# Autodesk Inventor assembly: OBG-Gehäuse
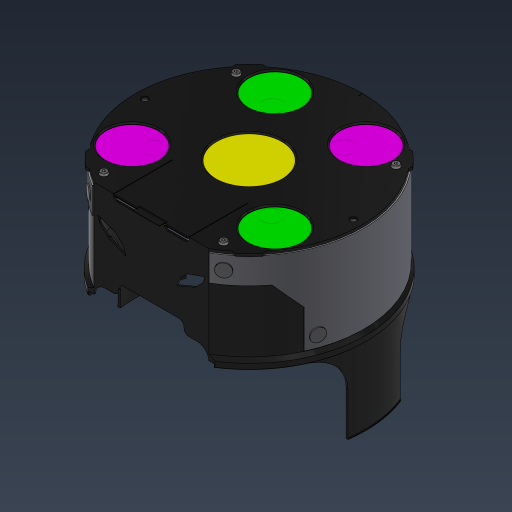
[picture p0: Inventor's stored thumbnail of the model, 512x512]
Saved by Autodesk Inventor 2023.1 (Build 271208000, 208)
## iProperties
Part Number: OBG-Gehäuse
Material: Generisch
Document SubType Name: Assembly
Designer: rYan
Mass: 129.127 g
Surface Area: 1997.42 cm^2
Volume: 130.879 cm^3
Density: 0.986618 g/cm^3
Author: rYan
## Documents named in this file (8)
- D:\TIGERsGIT\Hardware\mechanik\2024\Inventor\Robot\Case\OBG-Gehäuse.iam
- D:\TIGERsGIT\Hardware\mechanik\2024\Inventor\Robot\Case\Gehäuse Unterplatte.ipt
- D:\TIGERsGIT\Hardware\mechanik\2024\Inventor\Purchased Parts\Papier 40mm.ipt
- D:\TIGERsGIT\Hardware\mechanik\2024\Inventor\Inhaltscenter\de-DE\DIN 7984\DIN 7984 - M3 x 5.ipt
- D:\TIGERsGIT\Hardware\mechanik\2024\Inventor\Purchased Parts\Papier Teamfarbe.ipt
- D:\TIGERsGIT\Hardware\mechanik\2024\Inventor\Robot\Case\Gehäuse Mantel.ipt
- D:\TIGERsGIT\Hardware\mechanik\2024\Inventor\Robot\Case\Gehäuse Schnappfolie.ipt
- D:\TIGERsGIT\Hardware\mechanik\2024\Inventor\Robot\Case\Druckknopf.ipt
## Components (17 placed, 7 different names)
1. Gehäuse Mantel magnetisch:1 — Passend:9, Passend:10, Fluchtend:6, Einfügen:1, Einfügen:2, Einfügen:3, Einfügen:4, Passend:17, Einfügen:5, Einfügen:6, Einfügen:7, Einfügen:8, Einfügen:9, Passend:20
2. Gehäuse Unterplatte:1 — Einfügen:9, Fluchtend:7
3. Gehäuse Schnappfolie:1 — Passend:18, Passend:19, Passend:20, Passend:21, Passend:22, Passend:23, Passend:24, Passend:25, Passend:26, Passend:27, Passend:28, Passend:29, Passend:30
4. DIN 7984 M3 x 5:1 — Einfügen:6
5. DIN 7984 M3 x 5:2 — Einfügen:7
6. DIN 7984 M3 x 5:3 — Einfügen:8
7. DIN 7984 M3 x 5:4 — Einfügen:5
8. Papier 40mm:1 — Einfügen:3
9. Papier 40mm:2 — Einfügen:1
10. Papier 40mm:3 — Einfügen:2
11. Papier 40mm:4 — Einfügen:4
12. Papier Teamfarbe:1 — Fluchtend:2, Passend:17
13. Druckknopf:1 — Passend:21, Passend:22
14. Druckknopf:2 — Passend:26, Passend:30
15. Druckknopf:3 — Passend:25, Passend:29
16. Druckknopf:4 — Passend:24, Passend:28
17. Druckknopf:5 — Passend:23, Passend:27
## Relationships (28: Mate 16, Insert 9, Flush 3)
- Fluchtend:2 [Flush]: Papier Teamfarbe:1
- Passend:9 [Mate]: Gehäuse Mantel magnetisch:1
- Passend:10 [Mate]: Gehäuse Mantel magnetisch:1
- Fluchtend:6 [Flush]: Gehäuse Mantel magnetisch:1
- Einfügen:1 [Insert]: Gehäuse Mantel magnetisch:1 ↔ Papier 40mm:2
- Einfügen:2 [Insert]: Gehäuse Mantel magnetisch:1 ↔ Papier 40mm:3
- Einfügen:3 [Insert]: Gehäuse Mantel magnetisch:1 ↔ Papier 40mm:1
- Einfügen:4 [Insert]: Gehäuse Mantel magnetisch:1 ↔ Papier 40mm:4
- Passend:17 [Mate]: Gehäuse Mantel magnetisch:1 ↔ Papier Teamfarbe:1
- Einfügen:5 [Insert]: Gehäuse Mantel magnetisch:1 ↔ DIN 7984 M3 x 5:4
- Einfügen:6 [Insert]: Gehäuse Mantel magnetisch:1 ↔ DIN 7984 M3 x 5:1
- Einfügen:7 [Insert]: Gehäuse Mantel magnetisch:1 ↔ DIN 7984 M3 x 5:2
- Einfügen:8 [Insert]: Gehäuse Mantel magnetisch:1 ↔ DIN 7984 M3 x 5:3
- Einfügen:9 [Insert] (0.2 mm): Gehäuse Mantel magnetisch:1 ↔ Gehäuse Unterplatte:1
- Fluchtend:7 [Flush]: Gehäuse Unterplatte:1
- Passend:18 [Mate]: Gehäuse Schnappfolie:1
- Passend:19 [Mate]: Gehäuse Schnappfolie:1
- Passend:20 [Mate] (0.2 mm): Gehäuse Mantel magnetisch:1 ↔ Gehäuse Schnappfolie:1
- Passend:21 [Mate]: Gehäuse Schnappfolie:1 ↔ Druckknopf:1
- Passend:22 [Mate]: Gehäuse Schnappfolie:1 ↔ Druckknopf:1
- Passend:23 [Mate]: Gehäuse Schnappfolie:1 ↔ Druckknopf:5
- Passend:24 [Mate]: Gehäuse Schnappfolie:1 ↔ Druckknopf:4
- Passend:25 [Mate]: Gehäuse Schnappfolie:1 ↔ Druckknopf:3
- Passend:26 [Mate]: Gehäuse Schnappfolie:1 ↔ Druckknopf:2
- Passend:27 [Mate]: Gehäuse Schnappfolie:1 ↔ Druckknopf:5
- Passend:28 [Mate]: Gehäuse Schnappfolie:1 ↔ Druckknopf:4
- Passend:29 [Mate]: Gehäuse Schnappfolie:1 ↔ Druckknopf:3
- Passend:30 [Mate]: Gehäuse Schnappfolie:1 ↔ Druckknopf:2
